# Autodesk Inventor assembly: PCB104_Hermes_Module_Assembled_V1
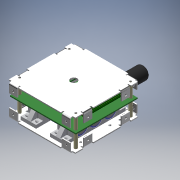
[picture p0: Inventor's stored thumbnail of the model, 180x180]
Saved by Autodesk Inventor 2017 (Build 210142000, 142)
## iProperties
Created: 2016-11-19
Part Number: PCB104_Hermes_Module_Assembled_V1
Document SubType Name: Assembly
Designer: Christopher
Author: Christopher
## Documents named in this file (12)
- C:\Users\qupec\Desktop\CADD\CADD\RSX Assembly\Hermes Cube.iam
- C:\Users\qupec\Desktop\CADD\CADD\RSX Assembly\Hermese Module\RPS Iridium 9603 SBD.ipt
- C:\Users\qupec\Desktop\CADD\CADD\RSX Assembly\Hermese Module\RapberryPiZero_Shrinkwrap_tomnappey.ipt
- C:\Users\qupec\Desktop\CADD\CADD\RSX Assembly\Hermese Module\RPS HERMES Mount.ipt
- C:\Users\qupec\Desktop\CADD\CADD\RSX Assembly\Hermese Module\RPS Long Spacer.ipt
- C:\Users\qupec\Desktop\CADD\CADD\RSX Assembly\Hermese Module\Short_Spacer_V1.ipt
- C:\Users\qupec\Desktop\CADD\CADD\RSX Assembly\Hermese Module\Med_Spacer_V1.ipt
- C:\Users\qupec\Desktop\CADD\CADD\RSX Assembly\Hermese Module\PC 104 size and hole model_Hermes_Top_Mount_V1.ipt
- C:\Users\qupec\Desktop\CADD\CADD\RSX Assembly\Hermese Module\RPS HERMES Antenna Mount side.ipt
- C:\Users\qupec\Desktop\CADD\CADD\RSX Assembly\Hermese Module\RPS Basic M3 Weld Nut.ipt
- C:\Users\qupec\Desktop\CADD\CADD\RSX Assembly\Hermese Module\ES Helix Antenna.ipt
- C:\Users\qupec\Desktop\CADD\CADD\RSX Assembly\Hermese Module\ES Battery 3 Cell.iam
## Components (37 placed, 11 different names)
1. RPS Iridium 9603 SBD:1 — Mate:38, Mate:39, Mate:40, Mate:41
2. RapberryPiZero_Shrinkwrap_tomnappey:1 — Mate:30, Mate:31, Mate:32, Mate:33, Mate:34, Mate:35, Mate:36, Mate:37
3. RPS HERMES Mount:1 — Insert:18, Insert:19, Insert:24, Insert:25, Insert:26, Insert:27, Insert:29, Insert:31, Insert:34, Insert:35, Mate:63, Flush:1, Flush:2
4. RPS HERMES Antenna Mount side:1 — Mate:42, Mate:43, Mate:44, Mate:45, Mate:46, Mate:47, Mate:48, Mate:49, Insert:20, Insert:21, Insert:22, Insert:23, Insert:28, Insert:30, Insert:32, Insert:33, Mate:66
5. RPS Long Spacer:1 — Insert:17, Insert:19
6. RPS Long Spacer:2 — Insert:14
7. RPS Long Spacer:3 — Insert:16
8. RPS Long Spacer:4 — Insert:15, Insert:18
9. Short_Spacer_V1:1 — Mate:34, Mate:35, Insert:12
10. Short_Spacer_V1:2 — Mate:36, Mate:37
11. Short_Spacer_V1:3 — Mate:32, Mate:33, Mate:60, Insert:13
12. Short_Spacer_V1:4 — Mate:30, Mate:31
13. Short_Spacer_V1:5 — Mate:38, Mate:39, Insert:11
14. Short_Spacer_V1:6 — Mate:40, Mate:41, Insert:10
15. Med_Spacer_V1:1 — Mate:48, Mate:49, Insert:9
16. Med_Spacer_V1:2 — Mate:42, Mate:43, Insert:8
17. Med_Spacer_V1:3 — Mate:46, Mate:47, Insert:6
18. Med_Spacer_V1:4 — Mate:44, Mate:45, Insert:7
19. PC 104 size and hole model_Hermes_Top_Mount_V1:1 — Mate:60, Insert:6, Insert:7, Insert:8, Insert:9, Insert:10, Insert:11, Insert:12, Insert:13, Insert:14, Insert:15, Insert:16, Insert:17, Mate:65
20. RPS Basic M3 Weld Nut:17 — Insert:28
21. RPS Basic M3 Weld Nut:18 — Insert:35
22. RPS Basic M3 Weld Nut:19 — Insert:21
23. RPS Basic M3 Weld Nut:20 — Insert:23
24. RPS Basic M3 Weld Nut:21 — Insert:26
25. RPS Basic M3 Weld Nut:22 — Insert:29
26. RPS Basic M3 Weld Nut:23 — Insert:33
27. RPS Basic M3 Weld Nut:24 — Insert:22
28. RPS Basic M3 Weld Nut:25 — Insert:20
29. RPS Basic M3 Weld Nut:26 — Insert:25
30. RPS Basic M3 Weld Nut:27 — Insert:27
31. RPS Basic M3 Weld Nut:28 — Insert:30
32. RPS Basic M3 Weld Nut:29 — Insert:32
33. RPS Basic M3 Weld Nut:30 — Insert:34
34. RPS Basic M3 Weld Nut:31 — Insert:24
35. RPS Basic M3 Weld Nut:32 — Insert:31
36. ES Helix Antenna:1 — Mate:65, Mate:66
37. ES Battery 3 Cell:1 [sub-assembly] — Mate:63, Flush:1, Flush:2
## Relationships (56: Insert 30, Mate 24, Flush 2)
- Mate:30: RapberryPiZero_Shrinkwrap_tomnappey:1 ↔ Short_Spacer_V1:4
- Mate:31: RapberryPiZero_Shrinkwrap_tomnappey:1 ↔ Short_Spacer_V1:4
- Mate:32: RapberryPiZero_Shrinkwrap_tomnappey:1 ↔ Short_Spacer_V1:3
- Mate:33: RapberryPiZero_Shrinkwrap_tomnappey:1 ↔ Short_Spacer_V1:3
- Mate:34: RapberryPiZero_Shrinkwrap_tomnappey:1 ↔ Short_Spacer_V1:1
- Mate:35: RapberryPiZero_Shrinkwrap_tomnappey:1 ↔ Short_Spacer_V1:1
- Mate:36: RapberryPiZero_Shrinkwrap_tomnappey:1 ↔ Short_Spacer_V1:2
- Mate:37: RapberryPiZero_Shrinkwrap_tomnappey:1 ↔ Short_Spacer_V1:2
- Mate:38: RPS Iridium 9603 SBD:1 ↔ Short_Spacer_V1:5
- Mate:39: RPS Iridium 9603 SBD:1 ↔ Short_Spacer_V1:5
- Mate:40: RPS Iridium 9603 SBD:1 ↔ Short_Spacer_V1:6
- Mate:41: RPS Iridium 9603 SBD:1 ↔ Short_Spacer_V1:6
- Mate:42: RPS HERMES Antenna Mount side:1 ↔ Med_Spacer_V1:2
- Mate:43: RPS HERMES Antenna Mount side:1 ↔ Med_Spacer_V1:2
- Mate:44: RPS HERMES Antenna Mount side:1 ↔ Med_Spacer_V1:4
- Mate:45: RPS HERMES Antenna Mount side:1 ↔ Med_Spacer_V1:4
- Mate:46: RPS HERMES Antenna Mount side:1 ↔ Med_Spacer_V1:3
- Mate:47: RPS HERMES Antenna Mount side:1 ↔ Med_Spacer_V1:3
- Mate:48: RPS HERMES Antenna Mount side:1 ↔ Med_Spacer_V1:1
- Mate:49: RPS HERMES Antenna Mount side:1 ↔ Med_Spacer_V1:1
- Mate:60: Short_Spacer_V1:3 ↔ PC 104 size and hole model_Hermes_Top_Mount_V1:1
- Insert:6: Med_Spacer_V1:3 ↔ PC 104 size and hole model_Hermes_Top_Mount_V1:1
- Insert:7: Med_Spacer_V1:4 ↔ PC 104 size and hole model_Hermes_Top_Mount_V1:1
- Insert:8: Med_Spacer_V1:2 ↔ PC 104 size and hole model_Hermes_Top_Mount_V1:1
- Insert:9: Med_Spacer_V1:1 ↔ PC 104 size and hole model_Hermes_Top_Mount_V1:1
- Insert:10: Short_Spacer_V1:6 ↔ PC 104 size and hole model_Hermes_Top_Mount_V1:1
- Insert:11: Short_Spacer_V1:5 ↔ PC 104 size and hole model_Hermes_Top_Mount_V1:1
- Insert:12: Short_Spacer_V1:1 ↔ PC 104 size and hole model_Hermes_Top_Mount_V1:1
- Insert:13: Short_Spacer_V1:3 ↔ PC 104 size and hole model_Hermes_Top_Mount_V1:1
- Insert:14: RPS Long Spacer:2 ↔ PC 104 size and hole model_Hermes_Top_Mount_V1:1
- Insert:15: RPS Long Spacer:4 ↔ PC 104 size and hole model_Hermes_Top_Mount_V1:1
- Insert:16: RPS Long Spacer:3 ↔ PC 104 size and hole model_Hermes_Top_Mount_V1:1
- Insert:17: RPS Long Spacer:1 ↔ PC 104 size and hole model_Hermes_Top_Mount_V1:1
- Insert:18: RPS HERMES Mount:1 ↔ RPS Long Spacer:4
- Insert:19: RPS HERMES Mount:1 ↔ RPS Long Spacer:1
- Insert:20: RPS HERMES Antenna Mount side:1 ↔ RPS Basic M3 Weld Nut:25
- Insert:21: RPS HERMES Antenna Mount side:1 ↔ RPS Basic M3 Weld Nut:19
- Insert:22: RPS HERMES Antenna Mount side:1 ↔ RPS Basic M3 Weld Nut:24
- Insert:23: RPS HERMES Antenna Mount side:1 ↔ RPS Basic M3 Weld Nut:20
- Insert:24: RPS HERMES Mount:1 ↔ RPS Basic M3 Weld Nut:31
- Insert:25: RPS HERMES Mount:1 ↔ RPS Basic M3 Weld Nut:26
- Insert:26: RPS HERMES Mount:1 ↔ RPS Basic M3 Weld Nut:21
- Insert:27: RPS HERMES Mount:1 ↔ RPS Basic M3 Weld Nut:27
- Insert:28: RPS HERMES Antenna Mount side:1 ↔ RPS Basic M3 Weld Nut:17
- Insert:29: RPS HERMES Mount:1 ↔ RPS Basic M3 Weld Nut:22
- Insert:30: RPS HERMES Antenna Mount side:1 ↔ RPS Basic M3 Weld Nut:28
- Insert:31: RPS HERMES Mount:1 ↔ RPS Basic M3 Weld Nut:32
- Insert:32: RPS HERMES Antenna Mount side:1 ↔ RPS Basic M3 Weld Nut:29
- Insert:33: RPS HERMES Antenna Mount side:1 ↔ RPS Basic M3 Weld Nut:23
- Insert:34: RPS HERMES Mount:1 ↔ RPS Basic M3 Weld Nut:30
- Insert:35: RPS HERMES Mount:1 ↔ RPS Basic M3 Weld Nut:18
- Mate:63: RPS HERMES Mount:1 ↔ ES Battery 3 Cell:1
- Flush:1 (-5.2451 mm): RPS HERMES Mount:1 ↔ ES Battery 3 Cell:1
- Flush:2 (16.002 mm): RPS HERMES Mount:1 ↔ ES Battery 3 Cell:1
- Mate:65 (13.97 mm): PC 104 size and hole model_Hermes_Top_Mount_V1:1 ↔ ES Helix Antenna:1
- Mate:66: RPS HERMES Antenna Mount side:1 ↔ ES Helix Antenna:1
